# Autodesk Inventor assembly: Shooter Assembly
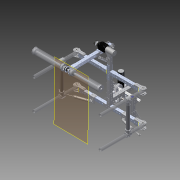
[picture p0: Inventor's stored thumbnail of the model, 180x180]
Saved by Autodesk Inventor 2014 SP1 (Build 180222100, 222)
## iProperties
Created: 2014-01-05
Part Number: Shooter Assembly
Document SubType Name: Assembly
Designer: Andrew Toennies
Mass: 10533.5 g
Surface Area: 21094.1 cm^2
Volume: 2538.58 cm^3
Density: 4.14937 g/cm^3
Author: Andrew Toennies
## Documents named in this file (33)
- C:\Users\Arpan\Documents\GitHub\2014buildCAD\Shooter\Shooter v1 (Defunct)\Shooter Assembly.iam
- C:\Users\Arpan\Documents\GitHub\2014buildCAD\Shooter\Shooter v1 (Defunct)\Vex Pro 1x1 rectangular tubing 12 in length.ipt
- C:\Users\Arpan\Documents\GitHub\2014buildCAD\Shooter\Shooter v1 (Defunct)\Vex Pro End Bearing Mount.ipt
- C:\Users\Arpan\Documents\GitHub\2014buildCAD\Shooter\Shooter v1 (Defunct)\Vex Pro 1x1 rectangular tubing 27 in length.ipt
- C:\Users\Arpan\Documents\GitHub\2014buildCAD\Shooter\Shooter v1 (Defunct)\Vex Pro Corner Gusset.ipt
- C:\Users\Arpan\Documents\GitHub\2014buildCAD\Shooter\Shooter v1 (Defunct)\Bearing ID 0.500 Hex OD 1.125.ipt
- C:\Users\Arpan\Documents\GitHub\2014buildCAD\Shooter\Shooter v1 (Defunct)\Spacer.ipt
- C:\Users\Arpan\Documents\GitHub\2014buildCAD\Shooter\Shooter v1 (Defunct)\Bearing ID 0.375 OD 1.125.ipt
- C:\Users\Arpan\Documents\GitHub\2014buildCAD\Shooter\Shooter v1 (Defunct)\Axle 0.375 3 in length.ipt
- C:\Users\Arpan\Documents\GitHub\2014buildCAD\Shooter\Shooter v1 (Defunct)\Axle 0.500 Hex 3 in length.ipt
- C:\Users\Arpan\Documents\GitHub\2014buildCAD\Shooter\Shooter v1 (Defunct)\Worm-Drive-Gearbox-16to1.iam
- C:\Users\Arpan\Documents\GitHub\2014buildCAD\Shooter\Shooter v1 (Defunct)\Vex Pro 32 tooth 15 mm timing belt pulley.ipt
- C:\Users\Arpan\Documents\GitHub\2014buildCAD\Shooter\Shooter v1 (Defunct)\Foot Bracket Mount (McMaster Part #6498K710).ipt
- C:\Users\Arpan\Documents\GitHub\2014buildCAD\Shooter\Shooter v1 (Defunct)\Rod End (McMaster Part #6498K592).ipt
- C:\Users\Arpan\Documents\GitHub\2014buildCAD\Shooter\Shooter v1 (Defunct)\Spacer2.ipt
- C:\Users\Arpan\Documents\GitHub\2014buildCAD\Shooter\Shooter v1 (Defunct)\Bracket.ipt
- C:\Users\Arpan\Documents\GitHub\2014buildCAD\Shooter\Shooter v1 (Defunct)\Axle 0.190 in 3 in length.ipt
- C:\Users\Arpan\Documents\GitHub\2014buildCAD\Shooter\Shooter v1 (Defunct)\6498K602 Pneumatic Cylinder Assembly.iam
- C:\Users\Arpan\Documents\GitHub\2014buildCAD\Shooter\Shooter v1 (Defunct)\mcmaster carr 32 tooth pulley.ipt
- C:\Users\Arpan\Documents\GitHub\2014buildCAD\Shooter\Shooter v1 (Defunct)\Vex Pro 1x1 rectangular tubing 4 in length.ipt
- C:\Users\Arpan\Documents\GitHub\2014buildCAD\Shooter\Shooter v1 (Defunct)\Vex Pro VersaFrame 90 Degree.ipt
- C:\Users\Arpan\Documents\GitHub\2014buildCAD\Shooter\Shooter v1 (Defunct)\Vex Pro Side Bearing Gusset.ipt
- C:\Users\Arpan\Documents\GitHub\2014buildCAD\Shooter\Shooter v1 (Defunct)\Steel Plate (0.0625).ipt
- C:\Users\Arpan\Documents\GitHub\2014buildCAD\Collector\Drive Roller Assembly.iam
- C:\Users\Arpan\Documents\GitHub\2014buildCAD\Shooter\Shooter v1 (Defunct)\Vex Pro 1x1 rectangular tubing 7 in length.ipt
- C:\Users\Arpan\Documents\GitHub\2014buildCAD\Shooter\Shooter v1 (Defunct)\Vex Pro T gusset.ipt
- C:\Users\Arpan\Documents\GitHub\2014buildCAD\Collector\Clamp with Piston Assembly.iam
- C:\Users\Arpan\Documents\GitHub\2014buildCAD\Shooter\Shooter v1 (Defunct)\Vex Pro Plus Gusset.ipt
- C:\Users\Arpan\Documents\GitHub\2014buildCAD\Collector\Piston Assembly.iam
- C:\Users\Arpan\Documents\GitHub\2014buildCAD\Collector\Pneumatic Piston Back Flange (Left Custom).ipt
- C:\Users\Arpan\Documents\GitHub\2014buildCAD\Collector\Pneumatic Piston Back Flange (Right Custom).ipt
- C:\Users\Arpan\Documents\GitHub\2014buildCAD\Shooter\Shooter v1 (Defunct)\Vex Pro 1x1 rectangular tubing 23 in length.ipt
- C:\Users\Arpan\Documents\GitHub\2014buildCAD\Shooter\Shooter v1 (Defunct)\Spacer 3.ipt
## Components (77 placed, 32 different names)
1. Vex Pro Corner Gusset:1 — Insert:9, Insert:10, Flush:60, Flush:61
2. Vex Pro Corner Gusset:2 — Insert:11, Insert:12, Mate:261, Mate:262
3. Vex Pro End Bearing Mount:3 — Insert:116, Insert:117, Insert:118
4. Vex Pro End Bearing Mount:4 — Insert:36, Insert:49, Insert:50
5. Spacer:1 — Insert:114, Insert:115, Insert:116, Insert:117
6. Spacer:2 — Insert:49, Insert:50, Insert:112, Insert:113
7. Bearing ID 0.375 OD 1.125:1 — Mate:9, Insert:118, Flush:94
8. Bearing ID 0.375 OD 1.125:2 — Insert:36, Mate:66
9. Axle 0.375 3 in length:1 — Mate:9, Mate:66, Mate:269, Flush:94
10. Axle 0.500 Hex 3 in length:1 — Mate:47, Mate:48, Mate:210, Mate:211, Flush:59, Mate:250, Mate:251, Mate:258, Mate:259
11. Worm-Drive-Gearbox-16to1:1 [sub-assembly] — Mate:49, Mate:50, Mate:170, Mate:196, Mate:249
12. Vex Pro 32 tooth 15 mm timing belt pulley:1 — Mate:47, Mate:48, Flush:40, Rotation:1
13. Foot Bracket Mount (McMaster Part #6498K710):1 — Mate:71, Mate:72, Mate:73, Mate:99, Mate:100
14. Rod End (McMaster Part #6498K592):1 — Mate:103, Mate:326
15. Spacer2:1 — Mate:71, Mate:72, Mate:73, Mate:315, Insert:131
16. Bracket:1 — Mate:96, Flush:25, Mate:275, Mate:276, Insert:130
17. Bracket:2 — Mate:97, Mate:270, Mate:273, Mate:274
18. Axle 0.190 in 3 in length:1 — Mate:96, Mate:97, Flush:25, Mate:103
19. 6498K602 Pneumatic Cylinder Assembly:1 [sub-assembly] — Mate:99, Mate:100, Mate:326
20. mcmaster carr 32 tooth pulley:1 — Mate:170, Flush:40, Rotation:1, Mate:249, Flush:85
21. Bearing ID 0.500 Hex OD 1.125:4 — Flush:57, Mate:210, Flush:59, Insert:68
22. Bearing ID 0.500 Hex OD 1.125:3 — Insert:67
23. Bearing ID 0.500 Hex OD 1.125:7 — Flush:57, Mate:211, Insert:65, Flush:86
24. Vex Pro Corner Gusset:9 — Flush:60, Flush:61, Flush:64, Flush:65, Mate:218, Flush:66, Flush:67
25. Vex Pro Corner Gusset:10 — Flush:64, Flush:65, Mate:219, Mate:262
26. Vex Pro Side Bearing Gusset:1 — Mate:232, Mate:233, Mate:234, Insert:68
27. Vex Pro Side Bearing Gusset:2 — Mate:235, Mate:236, Mate:237, Insert:65
28. Vex Pro Side Bearing Gusset:3 — Mate:238, Mate:239, Mate:240, Insert:70
29. Vex Pro Side Bearing Gusset:4 — Mate:241, Mate:242, Mate:243, Insert:67
30. Vex Pro VersaFrame 90 Degree:1 — Mate:254, Insert:122, Mate:328, Mate:329
31. Vex Pro VersaFrame 90 Degree:2 — Insert:127, Insert:128, Mate:330
32. Vex Pro 32 tooth 15 mm timing belt pulley:2 — Mate:258, Mate:259, Flush:85
33. Bearing ID 0.500 Hex OD 1.125:8 — Insert:70, Flush:86
34. Steel Plate (0.0625):1 — Mate:263, Mate:264, Mate:265
35. Steel Plate (0.0625):2 — Mate:266, Mate:267, Mate:268
36. Drive Roller Assembly:1 [sub-assembly] — Mate:269, Mate:270, Mate:273, Mate:274, Mate:275, Mate:276, Flush:92, Insert:130
37. Vex Pro 1x1 rectangular tubing 7 in length:1 — Flush:89, Insert:108, Insert:109, Insert:126, Insert:192, Insert:193, Insert:194, Insert:195
38. Vex Pro 1x1 rectangular tubing 7 in length:2 — Flush:89, Insert:104, Insert:105, Insert:125, Insert:184, Insert:185, Insert:186, Insert:187
39. Vex Pro T gusset:1 — Insert:123, Insert:124, Insert:125, Insert:126
40. Clamp with Piston Assembly:2 [sub-assembly] — Mate:319, Angle:3, Mate:331, Mate:332
41. Vex Pro Plus Gusset:1 — Insert:81, Insert:121, Insert:166, Insert:167
42. Vex Pro Plus Gusset:2 — Insert:83, Insert:84, Insert:129
43. Piston Assembly:1 [sub-assembly] — Insert:106, Insert:107
44. Piston Assembly:2 [sub-assembly] — Insert:110, Insert:111
45. Pneumatic Piston Back Flange (Left Custom):1 — Insert:104, Insert:105, Insert:106, Insert:107
46. Pneumatic Piston Back Flange (Right Custom):1 — Insert:108, Insert:109, Insert:110, Insert:111
47. Spacer 3:1 — Insert:134, Insert:135, Insert:180, Insert:181
48. Vex Pro End Bearing Mount:13 — Insert:134, Insert:135, Insert:176
49. Spacer 3:3 — Insert:182, Insert:183
50. Vex Pro End Bearing Mount:14 — Insert:177, Mate:333
51. Spacer 3:4 — Insert:184, Insert:185
52. Vex Pro End Bearing Mount:15 — Insert:179
53. Spacer 3:5 — Insert:186, Insert:187
54. Vex Pro End Bearing Mount:16 — Insert:178, Mate:334
55. Spacer 3:6 — Insert:190, Insert:191
56. Vex Pro End Bearing Mount:17 — Insert:173, Mate:332
57. Spacer 3:7 — Insert:188, Insert:189
58. Vex Pro End Bearing Mount:18 — Insert:172
59. Spacer 3:8 — Insert:194, Insert:195
60. Vex Pro End Bearing Mount:19 — Mate:319, Insert:175, Mate:331
61. Spacer 3:9 — Insert:192, Insert:193
62. Vex Pro End Bearing Mount:20 — Insert:174
63. Vex Pro 1x1 rectangular tubing 7 in length:5 — Insert:166, Insert:167, Angle:3, Insert:188, Insert:189, Insert:190, Insert:191
64. Bearing ID 0.375 OD 1.125:3 — Insert:173
65. Bearing ID 0.375 OD 1.125:4 — Insert:172
66. Bearing ID 0.375 OD 1.125:5 — Insert:175
67. Bearing ID 0.375 OD 1.125:6 — Insert:174
68. Bearing ID 0.375 OD 1.125:7 — Insert:176, Mate:335
69. Bearing ID 0.375 OD 1.125:8 — Insert:177
70. Bearing ID 0.375 OD 1.125:9 — Insert:178
71. Bearing ID 0.375 OD 1.125:10 — Insert:179, Mate:336
72. Clamp with Piston Assembly:3 [sub-assembly] — Mate:333, Mate:334, Mate:335, Mate:336
73. Vex Pro 1x1 rectangular tubing 7 in length:4 — Insert:81, Insert:83, Insert:84, Insert:180, Insert:181, Insert:182, Insert:183
74. Vex Pro 1x1 rectangular tubing 23 in length:1 — Insert:112, Insert:113, Insert:114, Insert:115, Flush:92, Insert:121, Insert:122, Insert:123, Insert:124, Insert:127, Insert:128, Insert:129, Mate:315, Insert:131, Mate:328
75. Vex Pro 1x1 rectangular tubing 4 in length:1 — Mate:218, Flush:66, Flush:67, Mate:219, Mate:235, Mate:236, Mate:237, Mate:238, Mate:239, Mate:240, Angle:1
76. Vex Pro 1x1 rectangular tubing 12 in length:1 — Insert:9, Insert:10, Insert:11, Insert:12, Mate:49, Mate:50, Mate:196, Mate:232, Mate:233, Mate:234, Mate:241, Mate:242, Mate:243
77. Vex Pro 1x1 rectangular tubing 27 in length:1 — Mate:250, Mate:251, Mate:254, Mate:261, Mate:263, Mate:264, Mate:265, Mate:266, Mate:267, Mate:268, Angle:1, Mate:329, Mate:330
## Relationships (164: Insert 82, Mate 64, Flush 15, Angle 2, RelateRotation 1)
- Insert:9: Vex Pro Corner Gusset:1 ↔ Vex Pro 1x1 rectangular tubing 12 in length:1
- Insert:10: Vex Pro Corner Gusset:1 ↔ Vex Pro 1x1 rectangular tubing 12 in length:1
- Insert:11: Vex Pro Corner Gusset:2 ↔ Vex Pro 1x1 rectangular tubing 12 in length:1
- Insert:12: Vex Pro Corner Gusset:2 ↔ Vex Pro 1x1 rectangular tubing 12 in length:1
- Insert:36: Vex Pro End Bearing Mount:4 ↔ Bearing ID 0.375 OD 1.125:2
- Mate:9: Bearing ID 0.375 OD 1.125:1 ↔ Axle 0.375 3 in length:1
- Mate:47: Axle 0.500 Hex 3 in length:1 ↔ Vex Pro 32 tooth 15 mm timing belt pulley:1
- Mate:48: Axle 0.500 Hex 3 in length:1 ↔ Vex Pro 32 tooth 15 mm timing belt pulley:1
- Mate:49: Worm-Drive-Gearbox-16to1:1 ↔ Vex Pro 1x1 rectangular tubing 12 in length:1
- Mate:50: Worm-Drive-Gearbox-16to1:1 ↔ Vex Pro 1x1 rectangular tubing 12 in length:1
- Insert:49: Vex Pro End Bearing Mount:4 ↔ Spacer:2
- Insert:50: Vex Pro End Bearing Mount:4 ↔ Spacer:2
- Mate:66: Bearing ID 0.375 OD 1.125:2 ↔ Axle 0.375 3 in length:1
- Mate:71: Foot Bracket Mount (McMaster Part #6498K710):1 ↔ Spacer2:1
- Mate:72: Foot Bracket Mount (McMaster Part #6498K710):1 ↔ Spacer2:1
- Mate:73: Foot Bracket Mount (McMaster Part #6498K710):1 ↔ Spacer2:1
- Mate:96: Bracket:1 ↔ Axle 0.190 in 3 in length:1
- Mate:97: Bracket:2 ↔ Axle 0.190 in 3 in length:1
- Flush:25 (-11.1125 mm): Bracket:1 ↔ Axle 0.190 in 3 in length:1
- Mate:99: Foot Bracket Mount (McMaster Part #6498K710):1 ↔ 6498K602 Pneumatic Cylinder Assembly:1
- Mate:100: Foot Bracket Mount (McMaster Part #6498K710):1 ↔ 6498K602 Pneumatic Cylinder Assembly:1
- Mate:103: Rod End (McMaster Part #6498K592):1 ↔ Axle 0.190 in 3 in length:1
- Mate:170: Worm-Drive-Gearbox-16to1:1 ↔ mcmaster carr 32 tooth pulley:1
- Flush:40: Vex Pro 32 tooth 15 mm timing belt pulley:1 ↔ mcmaster carr 32 tooth pulley:1
- Rotation:1 [RelateRotation] (1 ul): Vex Pro 32 tooth 15 mm timing belt pulley:1 ↔ mcmaster carr 32 tooth pulley:1
- Mate:196: Worm-Drive-Gearbox-16to1:1 ↔ Vex Pro 1x1 rectangular tubing 12 in length:1
- Flush:57: Bearing ID 0.500 Hex OD 1.125:4 ↔ Bearing ID 0.500 Hex OD 1.125:7
- Mate:210: Axle 0.500 Hex 3 in length:1 ↔ Bearing ID 0.500 Hex OD 1.125:4
- Mate:211: Axle 0.500 Hex 3 in length:1 ↔ Bearing ID 0.500 Hex OD 1.125:7
- Flush:59 (12.7 mm): Axle 0.500 Hex 3 in length:1 ↔ Bearing ID 0.500 Hex OD 1.125:4
- Flush:60: Vex Pro Corner Gusset:1 ↔ Vex Pro Corner Gusset:9
- Flush:61: Vex Pro Corner Gusset:1 ↔ Vex Pro Corner Gusset:9
- Flush:64: Vex Pro Corner Gusset:9 ↔ Vex Pro Corner Gusset:10
- Flush:65: Vex Pro Corner Gusset:9 ↔ Vex Pro Corner Gusset:10
- Mate:218: Vex Pro Corner Gusset:9 ↔ Vex Pro 1x1 rectangular tubing 4 in length:1
- Flush:66: Vex Pro Corner Gusset:9 ↔ Vex Pro 1x1 rectangular tubing 4 in length:1
- Flush:67: Vex Pro Corner Gusset:9 ↔ Vex Pro 1x1 rectangular tubing 4 in length:1
- Mate:219: Vex Pro Corner Gusset:10 ↔ Vex Pro 1x1 rectangular tubing 4 in length:1
- Mate:232: Vex Pro Side Bearing Gusset:1 ↔ Vex Pro 1x1 rectangular tubing 12 in length:1
- Mate:233: Vex Pro Side Bearing Gusset:1 ↔ Vex Pro 1x1 rectangular tubing 12 in length:1
- Mate:234: Vex Pro Side Bearing Gusset:1 ↔ Vex Pro 1x1 rectangular tubing 12 in length:1
- Mate:235: Vex Pro Side Bearing Gusset:2 ↔ Vex Pro 1x1 rectangular tubing 4 in length:1
- Mate:236: Vex Pro Side Bearing Gusset:2 ↔ Vex Pro 1x1 rectangular tubing 4 in length:1
- Mate:237: Vex Pro Side Bearing Gusset:2 ↔ Vex Pro 1x1 rectangular tubing 4 in length:1
- Mate:238: Vex Pro Side Bearing Gusset:3 ↔ Vex Pro 1x1 rectangular tubing 4 in length:1
- Mate:239: Vex Pro Side Bearing Gusset:3 ↔ Vex Pro 1x1 rectangular tubing 4 in length:1
- Mate:240: Vex Pro Side Bearing Gusset:3 ↔ Vex Pro 1x1 rectangular tubing 4 in length:1
- Mate:241: Vex Pro Side Bearing Gusset:4 ↔ Vex Pro 1x1 rectangular tubing 12 in length:1
- Mate:242: Vex Pro Side Bearing Gusset:4 ↔ Vex Pro 1x1 rectangular tubing 12 in length:1
- Mate:243: Vex Pro Side Bearing Gusset:4 ↔ Vex Pro 1x1 rectangular tubing 12 in length:1
- Insert:65: Bearing ID 0.500 Hex OD 1.125:7 ↔ Vex Pro Side Bearing Gusset:2
- Insert:67: Bearing ID 0.500 Hex OD 1.125:3 ↔ Vex Pro Side Bearing Gusset:4
- Insert:68: Bearing ID 0.500 Hex OD 1.125:4 ↔ Vex Pro Side Bearing Gusset:1
- Mate:249 (12.7 mm): Worm-Drive-Gearbox-16to1:1 ↔ mcmaster carr 32 tooth pulley:1
- Mate:250: Axle 0.500 Hex 3 in length:1 ↔ Vex Pro 1x1 rectangular tubing 27 in length:1
- Mate:251: Axle 0.500 Hex 3 in length:1 ↔ Vex Pro 1x1 rectangular tubing 27 in length:1
- Mate:254: Vex Pro VersaFrame 90 Degree:1 ↔ Vex Pro 1x1 rectangular tubing 27 in length:1
- Mate:258: Axle 0.500 Hex 3 in length:1 ↔ Vex Pro 32 tooth 15 mm timing belt pulley:2
- Mate:259: Axle 0.500 Hex 3 in length:1 ↔ Vex Pro 32 tooth 15 mm timing belt pulley:2
- Flush:85: mcmaster carr 32 tooth pulley:1 ↔ Vex Pro 32 tooth 15 mm timing belt pulley:2
- Insert:70: Vex Pro Side Bearing Gusset:3 ↔ Bearing ID 0.500 Hex OD 1.125:8
- Flush:86: Bearing ID 0.500 Hex OD 1.125:7 ↔ Bearing ID 0.500 Hex OD 1.125:8
- Mate:261: Vex Pro Corner Gusset:2 ↔ Vex Pro 1x1 rectangular tubing 27 in length:1
- Mate:262 (31.75 mm): Vex Pro Corner Gusset:2 ↔ Vex Pro Corner Gusset:10
- Mate:263: Steel Plate (0.0625):1 ↔ Vex Pro 1x1 rectangular tubing 27 in length:1
- Mate:264: Steel Plate (0.0625):1 ↔ Vex Pro 1x1 rectangular tubing 27 in length:1
- Mate:265: Steel Plate (0.0625):1 ↔ Vex Pro 1x1 rectangular tubing 27 in length:1
- Mate:266: Steel Plate (0.0625):2 ↔ Vex Pro 1x1 rectangular tubing 27 in length:1
- Mate:267: Steel Plate (0.0625):2 ↔ Vex Pro 1x1 rectangular tubing 27 in length:1
- Mate:268: Steel Plate (0.0625):2 ↔ Vex Pro 1x1 rectangular tubing 27 in length:1
- Mate:269: Axle 0.375 3 in length:1 ↔ Drive Roller Assembly:1
- Mate:270: Bracket:2 ↔ Drive Roller Assembly:1
- Mate:273: Bracket:2 ↔ Drive Roller Assembly:1
- Mate:274: Bracket:2 ↔ Drive Roller Assembly:1
- Mate:275: Bracket:1 ↔ Drive Roller Assembly:1
- Mate:276: Bracket:1 ↔ Drive Roller Assembly:1
- Angle:1 (0 deg): Vex Pro 1x1 rectangular tubing 4 in length:1 ↔ Vex Pro 1x1 rectangular tubing 27 in length:1
- Flush:89: Vex Pro 1x1 rectangular tubing 7 in length:1 ↔ Vex Pro 1x1 rectangular tubing 7 in length:2
- Insert:81: Vex Pro Plus Gusset:1 ↔ Vex Pro 1x1 rectangular tubing 7 in length:4
- Insert:83: Vex Pro Plus Gusset:2 ↔ Vex Pro 1x1 rectangular tubing 7 in length:4
- Insert:84: Vex Pro Plus Gusset:2 ↔ Vex Pro 1x1 rectangular tubing 7 in length:4
- Insert:104: Vex Pro 1x1 rectangular tubing 7 in length:2 ↔ Pneumatic Piston Back Flange (Left Custom):1
- Insert:105: Vex Pro 1x1 rectangular tubing 7 in length:2 ↔ Pneumatic Piston Back Flange (Left Custom):1
- Insert:106: Piston Assembly:1 ↔ Pneumatic Piston Back Flange (Left Custom):1
- Insert:107: Piston Assembly:1 ↔ Pneumatic Piston Back Flange (Left Custom):1
- Insert:108: Vex Pro 1x1 rectangular tubing 7 in length:1 ↔ Pneumatic Piston Back Flange (Right Custom):1
- Insert:109: Vex Pro 1x1 rectangular tubing 7 in length:1 ↔ Pneumatic Piston Back Flange (Right Custom):1
- Insert:110: Piston Assembly:2 ↔ Pneumatic Piston Back Flange (Right Custom):1
- Insert:111: Piston Assembly:2 ↔ Pneumatic Piston Back Flange (Right Custom):1
- Insert:112: Spacer:2 ↔ Vex Pro 1x1 rectangular tubing 23 in length:1
- Insert:113: Spacer:2 ↔ Vex Pro 1x1 rectangular tubing 23 in length:1
- Insert:114: Spacer:1 ↔ Vex Pro 1x1 rectangular tubing 23 in length:1
- Insert:115: Spacer:1 ↔ Vex Pro 1x1 rectangular tubing 23 in length:1
- Insert:116: Vex Pro End Bearing Mount:3 ↔ Spacer:1
- Insert:117: Vex Pro End Bearing Mount:3 ↔ Spacer:1
- Insert:118: Vex Pro End Bearing Mount:3 ↔ Bearing ID 0.375 OD 1.125:1
- Flush:92: Drive Roller Assembly:1 ↔ Vex Pro 1x1 rectangular tubing 23 in length:1
- Insert:121: Vex Pro Plus Gusset:1 ↔ Vex Pro 1x1 rectangular tubing 23 in length:1
- Insert:122: Vex Pro VersaFrame 90 Degree:1 ↔ Vex Pro 1x1 rectangular tubing 23 in length:1
- Insert:123: Vex Pro T gusset:1 ↔ Vex Pro 1x1 rectangular tubing 23 in length:1
- Insert:124: Vex Pro T gusset:1 ↔ Vex Pro 1x1 rectangular tubing 23 in length:1
- Insert:125: Vex Pro 1x1 rectangular tubing 7 in length:2 ↔ Vex Pro T gusset:1
- Insert:126: Vex Pro 1x1 rectangular tubing 7 in length:1 ↔ Vex Pro T gusset:1
- Insert:127: Vex Pro VersaFrame 90 Degree:2 ↔ Vex Pro 1x1 rectangular tubing 23 in length:1
- Insert:128: Vex Pro VersaFrame 90 Degree:2 ↔ Vex Pro 1x1 rectangular tubing 23 in length:1
- Insert:129: Vex Pro Plus Gusset:2 ↔ Vex Pro 1x1 rectangular tubing 23 in length:1
- Mate:315: Spacer2:1 ↔ Vex Pro 1x1 rectangular tubing 23 in length:1
- Insert:130: Bracket:1 ↔ Drive Roller Assembly:1
- Insert:131: Spacer2:1 ↔ Vex Pro 1x1 rectangular tubing 23 in length:1
- Insert:134: Spacer 3:1 ↔ Vex Pro End Bearing Mount:13
- Insert:135: Spacer 3:1 ↔ Vex Pro End Bearing Mount:13
- [Insert]: Spacer 3:3 ↔ Vex Pro End Bearing Mount:14
- [Insert]: Spacer 3:3 ↔ Vex Pro End Bearing Mount:14
- [Insert]: Spacer 3:4 ↔ Vex Pro End Bearing Mount:15
- [Insert]: Spacer 3:4 ↔ Vex Pro End Bearing Mount:15
- [Insert]: Spacer 3:5 ↔ Vex Pro End Bearing Mount:16
- [Insert]: Spacer 3:5 ↔ Vex Pro End Bearing Mount:16
- [Insert]: Spacer 3:6 ↔ Vex Pro End Bearing Mount:17
- [Insert]: Spacer 3:6 ↔ Vex Pro End Bearing Mount:17
- [Insert]: Spacer 3:7 ↔ Vex Pro End Bearing Mount:18
- [Insert]: Spacer 3:7 ↔ Vex Pro End Bearing Mount:18
- [Insert]: Spacer 3:8 ↔ Vex Pro End Bearing Mount:19
- [Insert]: Spacer 3:8 ↔ Vex Pro End Bearing Mount:19
- [Insert]: Spacer 3:9 ↔ Vex Pro End Bearing Mount:20
- [Insert]: Spacer 3:9 ↔ Vex Pro End Bearing Mount:20
- Mate:319: Clamp with Piston Assembly:2 ↔ Vex Pro End Bearing Mount:19
- Insert:166: Vex Pro Plus Gusset:1 ↔ Vex Pro 1x1 rectangular tubing 7 in length:5
- Insert:167: Vex Pro Plus Gusset:1 ↔ Vex Pro 1x1 rectangular tubing 7 in length:5
- Insert:172: Vex Pro End Bearing Mount:18 ↔ Bearing ID 0.375 OD 1.125:4
- Insert:173: Vex Pro End Bearing Mount:17 ↔ Bearing ID 0.375 OD 1.125:3
- Insert:174: Vex Pro End Bearing Mount:20 ↔ Bearing ID 0.375 OD 1.125:6
- Insert:175: Vex Pro End Bearing Mount:19 ↔ Bearing ID 0.375 OD 1.125:5
- Insert:176: Vex Pro End Bearing Mount:13 ↔ Bearing ID 0.375 OD 1.125:7
- Insert:177: Vex Pro End Bearing Mount:14 ↔ Bearing ID 0.375 OD 1.125:8
- Insert:178: Vex Pro End Bearing Mount:16 ↔ Bearing ID 0.375 OD 1.125:9
- Insert:179: Vex Pro End Bearing Mount:15 ↔ Bearing ID 0.375 OD 1.125:10
- Mate:326: Rod End (McMaster Part #6498K592):1 ↔ 6498K602 Pneumatic Cylinder Assembly:1
- Angle:3 (270 deg): Clamp with Piston Assembly:2 ↔ Vex Pro 1x1 rectangular tubing 7 in length:5
- Insert:180: Spacer 3:1 ↔ Vex Pro 1x1 rectangular tubing 7 in length:4
- Insert:181: Spacer 3:1 ↔ Vex Pro 1x1 rectangular tubing 7 in length:4
- Insert:182: Spacer 3:3 ↔ Vex Pro 1x1 rectangular tubing 7 in length:4
- Insert:183: Spacer 3:3 ↔ Vex Pro 1x1 rectangular tubing 7 in length:4
- Insert:184: Vex Pro 1x1 rectangular tubing 7 in length:2 ↔ Spacer 3:4
- Insert:185: Vex Pro 1x1 rectangular tubing 7 in length:2 ↔ Spacer 3:4
- Insert:186: Vex Pro 1x1 rectangular tubing 7 in length:2 ↔ Spacer 3:5
- Insert:187: Vex Pro 1x1 rectangular tubing 7 in length:2 ↔ Spacer 3:5
- Insert:188: Spacer 3:7 ↔ Vex Pro 1x1 rectangular tubing 7 in length:5
- Insert:189: Spacer 3:7 ↔ Vex Pro 1x1 rectangular tubing 7 in length:5
- Insert:190: Spacer 3:6 ↔ Vex Pro 1x1 rectangular tubing 7 in length:5
- Insert:191: Spacer 3:6 ↔ Vex Pro 1x1 rectangular tubing 7 in length:5
- Insert:192: Vex Pro 1x1 rectangular tubing 7 in length:1 ↔ Spacer 3:9
- Insert:193: Vex Pro 1x1 rectangular tubing 7 in length:1 ↔ Spacer 3:9
- Insert:194: Vex Pro 1x1 rectangular tubing 7 in length:1 ↔ Spacer 3:8
- Insert:195: Vex Pro 1x1 rectangular tubing 7 in length:1 ↔ Spacer 3:8
- Mate:328: Vex Pro VersaFrame 90 Degree:1 ↔ Vex Pro 1x1 rectangular tubing 23 in length:1
- Mate:329: Vex Pro VersaFrame 90 Degree:1 ↔ Vex Pro 1x1 rectangular tubing 27 in length:1
- Mate:330: Vex Pro VersaFrame 90 Degree:2 ↔ Vex Pro 1x1 rectangular tubing 27 in length:1
- Flush:94 (-12.7 mm): Bearing ID 0.375 OD 1.125:1 ↔ Axle 0.375 3 in length:1
- Mate:331 (19.05 mm): Clamp with Piston Assembly:2 ↔ Vex Pro End Bearing Mount:19
- Mate:332 (19.05 mm): Clamp with Piston Assembly:2 ↔ Vex Pro End Bearing Mount:17
- Mate:333 (19.05 mm): Vex Pro End Bearing Mount:14 ↔ Clamp with Piston Assembly:3
- Mate:334 (19.05 mm): Vex Pro End Bearing Mount:16 ↔ Clamp with Piston Assembly:3
- Mate:335: Bearing ID 0.375 OD 1.125:7 ↔ Clamp with Piston Assembly:3
- Mate:336: Bearing ID 0.375 OD 1.125:10 ↔ Clamp with Piston Assembly:3
## Named parameters: d755_d751 = 0 mm, d756_d752 = 0 mm, d759_d755_d751 = 0 mm, d760_d756_d752 = 0 mm, d761_d755_d751 = 0 mm, d762_d756_d752 = 0 mm, d763_d755_d751 = 0 mm, d764_d756_d752 = 0 mm, d765_d755_d751 = 0 mm, d766_d756_d752 = 0 mm, d767_d755_d751 = 0 mm, d768_d756_d752 = 0 mm, d769_d755_d751 = 0 mm, d770_d756_d752 = 0 mm
